# Autodesk Inventor assembly: Engrenage_AX12
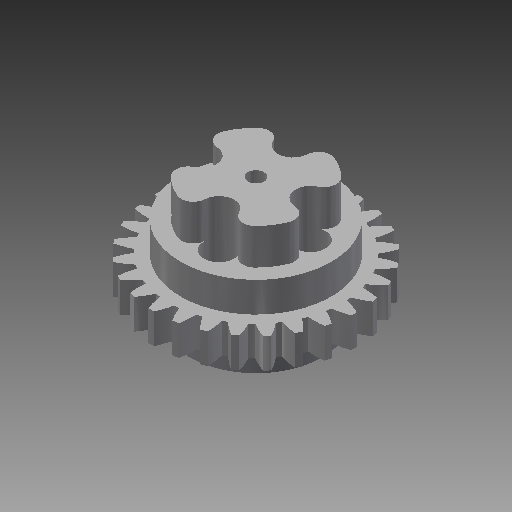
[picture p0: Inventor's stored thumbnail of the model, 512x512]
Saved by Autodesk Inventor 2018 (Build 220112000, 112)
## iProperties
Created: 2018-02-08
Part Number: Engrenage_AX12
Material: Générique
Document SubType Name: Assembly
Designer: Mephiro
Author: Mephiro
## Documents named in this file (3)
- C:\Users\Mephiro\Google Drive\Robot_cup_3D\Canon_v3\Engrenage_AX12.iam
- C:\Users\Mephiro\Google Drive\Robot_cup_3D\Canon_v3\Polonier AX.ipt
- C:\Users\Mephiro\Google Drive\Robot_cup_3D\Canon_v3\Engrenage_AX12\Design Accelerator\Engrenages cylindriques1.iam
## Components (2 placed, 2 different names)
1. Polonier AX:1 — Placage:1, Placage:2, Placage:3
2. Engrenages cylindriques:1 [sub-assembly] — Placage:1, Placage:2, Placage:3
## Relationships (3: Mate 3)
- Placage:1 [Mate]: Polonier AX:1 ↔ Engrenages cylindriques:1
- Placage:2 [Mate]: Polonier AX:1 ↔ Engrenages cylindriques:1
- Placage:3 [Mate]: Polonier AX:1 ↔ Engrenages cylindriques:1
